# Autodesk Inventor assembly: wall
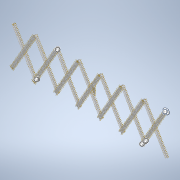
[picture p0: Inventor's stored thumbnail of the model, 180x180]
Saved by Autodesk Inventor 2020 (Build 240168000, 168)
## iProperties
Created: 2019-10-27
Part Number: wall
Document SubType Name: Assembly
Designer: Alex Zaccardelli
Author: Alex Zaccardelli
## Documents named in this file (5)
- D:\TrayBotCAD\wall.iam
- D:\TrayBotCAD\SIGBotsCADLibrary-20191023T040826Z-001\SIGBotsCADLibrary\SIGBotsCADLibrary\Structure\C-Channel 2 x 35 (aluminum).ipt
- D:\TrayBotCAD\SIGBotsCADLibrary-20191023T040826Z-001\SIGBotsCADLibrary\SIGBotsCADLibrary\Motion\Spacer 0.25 unit.ipt
- D:\TrayBotCAD\SIGBotsCADLibrary-20191023T040826Z-001\SIGBotsCADLibrary\SIGBotsCADLibrary\Motion\Spacer 1.0 unit.ipt
- D:\TrayBotCAD\SIGBotsCADLibrary-20191023T040826Z-001\SIGBotsCADLibrary\SIGBotsCADLibrary\Structure\C-Channel 5 x 5 (aluminum) Special.ipt
## Components (42 placed, 4 different names)
1. C-Channel 2 x 35 (aluminum):1 — Mate:4, Mate:5, Mate:6, Mate:7, Symmetry:1, Angle:2, Mate:22, Mate:23, Mate:32, Mate:33, Angle:10
2. Spacer 0.25 unit:1 — Mate:4, Mate:5, Mate:12, Mate:13
3. Spacer 1.0 unit:1 — Mate:6, Mate:7, Mate:8, Mate:9
4. Spacer 0.25 unit:2 — Mate:8, Mate:9, Mate:10, Mate:11
5. C-Channel 2 x 35 (aluminum):2 — Mate:10, Mate:11, Symmetry:1, Mate:18, Mate:19, Angle:3, Angle:5, Mate:74, Mate:75
6. C-Channel 5 x 5 (aluminum) Special:1 — Mate:12, Mate:13, Angle:1
7. C-Channel 2 x 35 (aluminum):3 — Mate:16, Mate:17, Angle:2, Mate:62, Mate:63, Angle:9
8. Spacer 1.0 unit:2 — Mate:16, Mate:17
9. Spacer 0.25 unit:3 — Mate:18, Mate:19
10. Spacer 1.0 unit:3 — Mate:23, Mate:24, Mate:25
11. Spacer 0.25 unit:4 — Mate:22
12. C-Channel 2 x 35 (aluminum):4 — Mate:24, Mate:25, Angle:3, Mate:58, Mate:59, Angle:8
13. Spacer 1.0 unit:5 — Mate:32, Mate:33, Mate:37
14. Spacer 0.25 unit:6 — Mate:36
15. C-Channel 2 x 35 (aluminum):6 — Mate:36, Mate:37, Angle:5, Angle:6, Mate:84, Mate:85
16. C-Channel 2 x 35 (aluminum):9 — Angle:6, Mate:68, Mate:69, Mate:94, Mate:95, Angle:14
17. Spacer 1.0 unit:10 — Mate:63, Mate:66, Mate:67
18. Spacer 0.25 unit:11 — Mate:62
19. Spacer 1.0 unit:11 — Mate:58, Mate:59, Mate:60, Mate:61
20. Spacer 0.25 unit:12 — Mate:60, Mate:61, Mate:64, Mate:65
21. C-Channel 2 x 35 (aluminum):10 — Mate:64, Mate:65, Angle:9, Mate:98, Mate:99, Angle:12
22. C-Channel 2 x 35 (aluminum):11 — Mate:66, Mate:67, Angle:8, Mate:102, Mate:103, Angle:13
23. C-Channel 2 x 35 (aluminum):12 — Mate:76, Mate:77, Mate:78, Mate:79, Angle:10, Angle:11
24. Spacer 0.25 unit:13 — Mate:68, Mate:69, Mate:70, Mate:71
25. Spacer 1.0 unit:12 — Mate:70, Mate:71, Mate:78, Mate:79
26. Spacer 1.0 unit:13 — Mate:72, Mate:73, Mate:74, Mate:75
27. Spacer 0.25 unit:14 — Mate:72, Mate:73, Mate:76, Mate:77
28. C-Channel 2 x 35 (aluminum):13 — Mate:86, Mate:87, Angle:11, Mate:92, Mate:93, Angle:15
29. Spacer 0.25 unit:15 — Mate:80, Mate:81, Mate:86
30. Spacer 1.0 unit:14 — Mate:80, Mate:81, Mate:84, Mate:85, Mate:87
31. Spacer 0.25 unit:16 — Mate:88, Mate:89, Mate:108
32. Spacer 1.0 unit:15 — Mate:88, Mate:89, Mate:92, Mate:93, Mate:109
33. Spacer 0.25 unit:17 — Mate:94, Mate:95
34. Spacer 1.0 unit:16 — Mate:110, Mate:111
35. Spacer 0.25 unit:18 — Mate:98, Mate:99
36. Spacer 1.0 unit:17 — Mate:106, Mate:107
37. Spacer 0.25 unit:19 — Mate:102
38. Spacer 1.0 unit:18 — Mate:103, Mate:104, Mate:105
39. C-Channel 2 x 35 (aluminum):14 — Mate:104, Mate:105, Angle:12
40. C-Channel 2 x 35 (aluminum):15 — Mate:106, Mate:107, Angle:13
41. C-Channel 2 x 35 (aluminum):16 — Mate:108, Mate:109, Angle:14
42. C-Channel 2 x 35 (aluminum):17 — Mate:110, Mate:111, Angle:15
## Relationships (96: Mate 82, Angle 13, Symmetry 1)
- Mate:4: C-Channel 2 x 35 (aluminum):1 ↔ Spacer 0.25 unit:1
- Mate:5: C-Channel 2 x 35 (aluminum):1 ↔ Spacer 0.25 unit:1
- Mate:6: C-Channel 2 x 35 (aluminum):1 ↔ Spacer 1.0 unit:1
- Mate:7: C-Channel 2 x 35 (aluminum):1 ↔ Spacer 1.0 unit:1
- Mate:8: Spacer 1.0 unit:1 ↔ Spacer 0.25 unit:2
- Mate:9: Spacer 1.0 unit:1 ↔ Spacer 0.25 unit:2
- Mate:10: Spacer 0.25 unit:2 ↔ C-Channel 2 x 35 (aluminum):2
- Mate:11: Spacer 0.25 unit:2 ↔ C-Channel 2 x 35 (aluminum):2
- Mate:12: Spacer 0.25 unit:1 ↔ C-Channel 5 x 5 (aluminum) Special:1
- Mate:13: Spacer 0.25 unit:1 ↔ C-Channel 5 x 5 (aluminum) Special:1
- Angle:1 (0 deg): C-Channel 5 x 5 (aluminum) Special:1
- Symmetry:1: C-Channel 2 x 35 (aluminum):1 ↔ C-Channel 2 x 35 (aluminum):2
- [Mate]: Spacer 1.0 unit:2 ↔ Spacer 0.25 unit:3
- [Mate]: Spacer 1.0 unit:2 ↔ Spacer 0.25 unit:3
- Mate:16: C-Channel 2 x 35 (aluminum):3 ↔ Spacer 1.0 unit:2
- Mate:17: C-Channel 2 x 35 (aluminum):3 ↔ Spacer 1.0 unit:2
- Mate:18: C-Channel 2 x 35 (aluminum):2 ↔ Spacer 0.25 unit:3
- Mate:19: C-Channel 2 x 35 (aluminum):2 ↔ Spacer 0.25 unit:3
- Angle:2 (0 deg): C-Channel 2 x 35 (aluminum):1 ↔ C-Channel 2 x 35 (aluminum):3
- [Mate]: Spacer 1.0 unit:3 ↔ Spacer 0.25 unit:4
- [Mate]: Spacer 1.0 unit:3 ↔ Spacer 0.25 unit:4
- Mate:22: C-Channel 2 x 35 (aluminum):1 ↔ Spacer 0.25 unit:4
- Mate:23: C-Channel 2 x 35 (aluminum):1 ↔ Spacer 1.0 unit:3
- Mate:24: Spacer 1.0 unit:3 ↔ C-Channel 2 x 35 (aluminum):4
- Mate:25: Spacer 1.0 unit:3 ↔ C-Channel 2 x 35 (aluminum):4
- Angle:3 (0 deg): C-Channel 2 x 35 (aluminum):2 ↔ C-Channel 2 x 35 (aluminum):4
- [Mate]: Spacer 1.0 unit:5 ↔ Spacer 0.25 unit:6
- [Mate]: Spacer 1.0 unit:5 ↔ Spacer 0.25 unit:6
- Mate:32: C-Channel 2 x 35 (aluminum):1 ↔ Spacer 1.0 unit:5
- Mate:33: C-Channel 2 x 35 (aluminum):1 ↔ Spacer 1.0 unit:5
- Mate:36: Spacer 0.25 unit:6 ↔ C-Channel 2 x 35 (aluminum):6
- Mate:37: Spacer 1.0 unit:5 ↔ C-Channel 2 x 35 (aluminum):6
- Angle:5 (0 deg): C-Channel 2 x 35 (aluminum):2 ↔ C-Channel 2 x 35 (aluminum):6
- Angle:6 (0 deg): C-Channel 2 x 35 (aluminum):6 ↔ C-Channel 2 x 35 (aluminum):9
- [Mate]: Spacer 1.0 unit:10 ↔ Spacer 0.25 unit:11
- [Mate]: Spacer 1.0 unit:10 ↔ Spacer 0.25 unit:11
- Mate:58: C-Channel 2 x 35 (aluminum):4 ↔ Spacer 1.0 unit:11
- Mate:59: C-Channel 2 x 35 (aluminum):4 ↔ Spacer 1.0 unit:11
- Mate:60: Spacer 1.0 unit:11 ↔ Spacer 0.25 unit:12
- Mate:61: Spacer 1.0 unit:11 ↔ Spacer 0.25 unit:12
- Mate:62: C-Channel 2 x 35 (aluminum):3 ↔ Spacer 0.25 unit:11
- Mate:63: C-Channel 2 x 35 (aluminum):3 ↔ Spacer 1.0 unit:10
- Mate:64: Spacer 0.25 unit:12 ↔ C-Channel 2 x 35 (aluminum):10
- Mate:65: Spacer 0.25 unit:12 ↔ C-Channel 2 x 35 (aluminum):10
- Mate:66: Spacer 1.0 unit:10 ↔ C-Channel 2 x 35 (aluminum):11
- Mate:67: Spacer 1.0 unit:10 ↔ C-Channel 2 x 35 (aluminum):11
- Angle:8 (0 deg): C-Channel 2 x 35 (aluminum):4 ↔ C-Channel 2 x 35 (aluminum):11
- Angle:9 (0 deg): C-Channel 2 x 35 (aluminum):3 ↔ C-Channel 2 x 35 (aluminum):10
- Mate:68: C-Channel 2 x 35 (aluminum):9 ↔ Spacer 0.25 unit:13
- Mate:69: C-Channel 2 x 35 (aluminum):9 ↔ Spacer 0.25 unit:13
- Mate:70: Spacer 0.25 unit:13 ↔ Spacer 1.0 unit:12
- Mate:71: Spacer 0.25 unit:13 ↔ Spacer 1.0 unit:12
- Mate:72: Spacer 1.0 unit:13 ↔ Spacer 0.25 unit:14
- Mate:73: Spacer 1.0 unit:13 ↔ Spacer 0.25 unit:14
- Mate:74: C-Channel 2 x 35 (aluminum):2 ↔ Spacer 1.0 unit:13
- Mate:75: C-Channel 2 x 35 (aluminum):2 ↔ Spacer 1.0 unit:13
- Mate:76: C-Channel 2 x 35 (aluminum):12 ↔ Spacer 0.25 unit:14
- Mate:77: C-Channel 2 x 35 (aluminum):12 ↔ Spacer 0.25 unit:14
- Mate:78: C-Channel 2 x 35 (aluminum):12 ↔ Spacer 1.0 unit:12
- Mate:79: C-Channel 2 x 35 (aluminum):12 ↔ Spacer 1.0 unit:12
- Angle:10 (0 deg): C-Channel 2 x 35 (aluminum):1 ↔ C-Channel 2 x 35 (aluminum):12
- Mate:80: Spacer 0.25 unit:15 ↔ Spacer 1.0 unit:14
- Mate:81: Spacer 0.25 unit:15 ↔ Spacer 1.0 unit:14
- Mate:84: C-Channel 2 x 35 (aluminum):6 ↔ Spacer 1.0 unit:14
- Mate:85: C-Channel 2 x 35 (aluminum):6 ↔ Spacer 1.0 unit:14
- Mate:86: C-Channel 2 x 35 (aluminum):13 ↔ Spacer 0.25 unit:15
- Mate:87: C-Channel 2 x 35 (aluminum):13 ↔ Spacer 1.0 unit:14
- Angle:11 (0 deg): C-Channel 2 x 35 (aluminum):12 ↔ C-Channel 2 x 35 (aluminum):13
- Mate:88: Spacer 0.25 unit:16 ↔ Spacer 1.0 unit:15
- Mate:89: Spacer 0.25 unit:16 ↔ Spacer 1.0 unit:15
- [Mate]: Spacer 0.25 unit:17 ↔ Spacer 1.0 unit:16
- [Mate]: Spacer 0.25 unit:17 ↔ Spacer 1.0 unit:16
- Mate:92: C-Channel 2 x 35 (aluminum):13 ↔ Spacer 1.0 unit:15
- Mate:93: C-Channel 2 x 35 (aluminum):13 ↔ Spacer 1.0 unit:15
- Mate:94: C-Channel 2 x 35 (aluminum):9 ↔ Spacer 0.25 unit:17
- Mate:95: C-Channel 2 x 35 (aluminum):9 ↔ Spacer 0.25 unit:17
- [Mate]: Spacer 0.25 unit:18 ↔ Spacer 1.0 unit:17
- [Mate]: Spacer 0.25 unit:18 ↔ Spacer 1.0 unit:17
- Mate:98: C-Channel 2 x 35 (aluminum):10 ↔ Spacer 0.25 unit:18
- Mate:99: C-Channel 2 x 35 (aluminum):10 ↔ Spacer 0.25 unit:18
- [Mate]: Spacer 0.25 unit:19 ↔ Spacer 1.0 unit:18
- [Mate]: Spacer 0.25 unit:19 ↔ Spacer 1.0 unit:18
- Mate:102: C-Channel 2 x 35 (aluminum):11 ↔ Spacer 0.25 unit:19
- Mate:103: C-Channel 2 x 35 (aluminum):11 ↔ Spacer 1.0 unit:18
- Mate:104: Spacer 1.0 unit:18 ↔ C-Channel 2 x 35 (aluminum):14
- Mate:105: Spacer 1.0 unit:18 ↔ C-Channel 2 x 35 (aluminum):14
- Angle:12 (0 deg): C-Channel 2 x 35 (aluminum):10 ↔ C-Channel 2 x 35 (aluminum):14
- Mate:106: Spacer 1.0 unit:17 ↔ C-Channel 2 x 35 (aluminum):15
- Mate:107: Spacer 1.0 unit:17 ↔ C-Channel 2 x 35 (aluminum):15
- Angle:13 (0 deg): C-Channel 2 x 35 (aluminum):11 ↔ C-Channel 2 x 35 (aluminum):15
- Mate:108: Spacer 0.25 unit:16 ↔ C-Channel 2 x 35 (aluminum):16
- Mate:109: Spacer 1.0 unit:15 ↔ C-Channel 2 x 35 (aluminum):16
- Angle:14 (0 deg): C-Channel 2 x 35 (aluminum):9 ↔ C-Channel 2 x 35 (aluminum):16
- Mate:110: Spacer 1.0 unit:16 ↔ C-Channel 2 x 35 (aluminum):17
- Mate:111: Spacer 1.0 unit:16 ↔ C-Channel 2 x 35 (aluminum):17
- Angle:15 (0 deg): C-Channel 2 x 35 (aluminum):13 ↔ C-Channel 2 x 35 (aluminum):17
## Named parameters: d14_d7 = 0 mm, d15_d8 = 0 mm, d21_d7 = 0 mm, d22_d8 = 0 mm, d32_d21_d7 = 0 mm, d33_d22_d8 = 0 mm, d62_d46_d32_d21_d7 = 0 mm, d63_d47_d33_d22_d8 = 0 mm, d103_d101 = 0 mm, d104_d102 = 0 mm, d109_d101 = 0 mm, d110_d102 = 0 mm, d113_d101 = 0 mm, d114_d102 = 0 mm
